# Autodesk Inventor assembly: Base
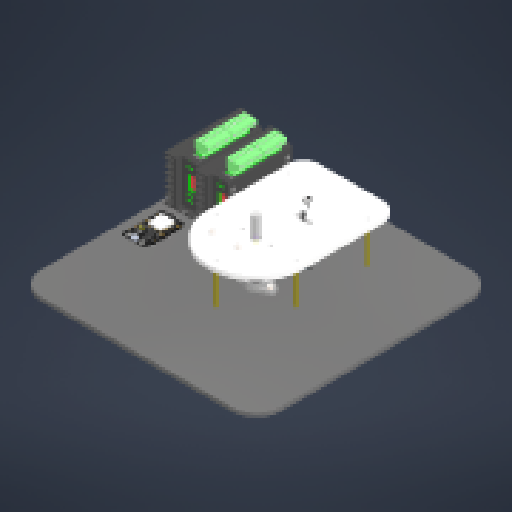
[picture p0: Inventor's stored thumbnail of the model, 512x512]
Saved by Autodesk Inventor 2023 (Build 270158000, 158)
## iProperties
Created: 2023-09-06
Part Number: Base
Document SubType Name: Assembly
Designer: philo
Sending System: Autodesk Inventor 2023
Preprocessor: ST-DEVELOPER v19
Title: C:\Users\philo\OneDrive\Desktop\HK1-2024\TT ROBOT\3DVer2\ROBOT_1_2.stp
Author: philo
## Documents named in this file (17)
- C:\Users\philo\OneDrive\Desktop\HK1-2024\TT ROBOT\02_3D_design_new\Base.iam
- C:\Users\philo\OneDrive\Desktop\HK1-2024\TT ROBOT\02_3D_design_new\DeRobot.ipt
- C:\Users\philo\OneDrive\Desktop\HK1-2024\TT ROBOT\02_3D_design_new\Detron.ipt
- C:\Users\philo\OneDrive\Desktop\HK1-2024\TT ROBOT\02_3D_design_new\goidoObi.ipt
- C:\Users\philo\OneDrive\Desktop\HK1-2024\TT ROBOT\02_3D_design_new\truday.ipt
- C:\Users\philo\OneDrive\Desktop\HK1-2024\TT ROBOT\02_3D_design_new\gt2_60teeth.iam
- C:\Users\philo\OneDrive\Desktop\HK1-2024\TT ROBOT\02_3D_design_new\M3 x 5mm.ipt
- C:\Users\philo\OneDrive\Desktop\HK1-2024\TT ROBOT\02_3D_design_new\Tb6600.ipt
- C:\Users\philo\OneDrive\Desktop\HK1-2024\TT ROBOT\02_3D_design_new\ESP-WROOM32.iam
- C:\Users\philo\OneDrive\Desktop\HK1-2024\TT ROBOT\02_3D_design_new\gt2smooth.ipt
- C:\Users\philo\OneDrive\Desktop\HK1-2024\TT ROBOT\02_3D_design_new\trudong5mm.ipt
- C:\Users\philo\OneDrive\Desktop\HK1-2024\TT ROBOT\02_3D_design_new\trucdogt2.ipt
- C:\Users\philo\OneDrive\Desktop\HK1-2024\TT ROBOT\02_3D_design_new\HALL.ipt
- C:\Users\philo\OneDrive\Desktop\HK1-2024\TT ROBOT\02_3D_design_new\namcham.ipt
- C:\Users\philo\OneDrive\Desktop\HK1-2024\TT ROBOT\02_3D_design_new\STEP MOTOR NEMA 17.ipt
- C:\Users\philo\OneDrive\Desktop\HK1-2024\TT ROBOT\02_3D_design_new\GT2 Pulley 20 Tooth (ID6mm).ipt
- C:\Users\philo\OneDrive\Desktop\HK1-2024\TT ROBOT\02_3D_design_new\oc5mm.ipt
## Components (28 placed, 16 different names)
1. oc5mm:4 — Mate:183, Mate:184
2. oc5mm:3 — Mate:182
3. oc5mm:2 — Mate:181
4. oc5mm:1 — Mate:179, Mate:180
5. GT2 Pulley 20 Tooth (ID6mm):1 — Mate:177, Mate:178
6. STEP MOTOR NEMA 17:1 — Mate:176, Flush:17, Flush:18, Mate:177
7. DeRobot:1 — Mate:81, Mate:82, Mate:83, Mate:84, Mate:85, Mate:86, Mate:87, Mate:90, Mate:91, Mate:92, Mate:95, Flush:16, Mate:174, Mate:175
8. Detron:1 — Mate:81, Mate:94, Mate:95, Mate:176, Flush:17, Flush:18, Mate:178, Mate:180, Mate:183
9. goidoObi:1 — Mate:93, Mate:94
10. goidoObi:2 — Mate:89, Mate:92
11. truday:1 — Mate:87, Mate:88, Mate:93, Flush:16
12. gt2_60teeth:1 [sub-assembly] — Mate:88, Mate:89
13. M3 x 5mm:1
14. M3 x 5mm:6
15. M3 x 5mm:7 — Mate:90
16. M3 x 5mm:8 — Mate:91
17. Tb6600:1 — Mate:174
18. Tb6600:2 — Mate:175
19. ESP-WROOM32:1 [sub-assembly]
20. gt2smooth:1 — Mate:99
21. trudong5mm:4 — Mate:84
22. trudong5mm:5 — Mate:82
23. trudong5mm:6 — Mate:85
24. trudong5mm:8 — Mate:86
25. trudong5mm:9 — Mate:83
26. trucdogt2:1 — Mate:99, Mate:179, Mate:181, Mate:182, Mate:184
27. HALL:1
28. namcham:1
## Relationships (30: Mate 27, Flush 3)
- Mate:81 (45 mm): DeRobot:1 ↔ Detron:1
- Mate:82: DeRobot:1 ↔ trudong5mm:5
- Mate:83: DeRobot:1 ↔ trudong5mm:9
- Mate:84: DeRobot:1 ↔ trudong5mm:4
- Mate:85: DeRobot:1 ↔ trudong5mm:6
- Mate:86: DeRobot:1 ↔ trudong5mm:8
- Mate:87: DeRobot:1 ↔ truday:1
- Mate:88: truday:1 ↔ gt2_60teeth:1
- Mate:89: goidoObi:2 ↔ gt2_60teeth:1
- Mate:90: DeRobot:1 ↔ M3 x 5mm:7
- Mate:91: DeRobot:1 ↔ M3 x 5mm:8
- Mate:92: DeRobot:1 ↔ goidoObi:2
- Mate:93: goidoObi:1 ↔ truday:1
- Mate:94: Detron:1 ↔ goidoObi:1
- Mate:95: DeRobot:1 ↔ Detron:1
- Mate:99: gt2smooth:1 ↔ trucdogt2:1
- Flush:16: DeRobot:1 ↔ truday:1
- Mate:174: DeRobot:1 ↔ Tb6600:1
- Mate:175: DeRobot:1 ↔ Tb6600:2
- Mate:176: STEP MOTOR NEMA 17:1 ↔ Detron:1
- Flush:17 (38 mm): STEP MOTOR NEMA 17:1 ↔ Detron:1
- Flush:18: STEP MOTOR NEMA 17:1 ↔ Detron:1
- Mate:177: GT2 Pulley 20 Tooth (ID6mm):1 ↔ STEP MOTOR NEMA 17:1
- Mate:178 (5 mm): GT2 Pulley 20 Tooth (ID6mm):1 ↔ Detron:1
- Mate:179: oc5mm:1 ↔ trucdogt2:1
- Mate:180: oc5mm:1 ↔ Detron:1
- Mate:181: oc5mm:2 ↔ trucdogt2:1
- Mate:182: oc5mm:3 ↔ trucdogt2:1
- Mate:183: oc5mm:4 ↔ Detron:1
- Mate:184: oc5mm:4 ↔ trucdogt2:1
